# Autodesk Inventor assembly: YIdlePulleyAssembly
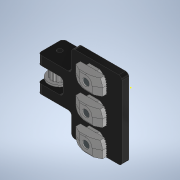
[picture p0: Inventor's stored thumbnail of the model, 180x180]
Saved by Autodesk Inventor 2020.2 (Build 242310000, 310)
## iProperties
Created: 2020-08-24
Part Number: YIdlePulleyAssembly
Document SubType Name: Assembly
Designer: JK
Author: JK
## Documents named in this file (5)
- C:\Users\JK\Documents\Inventor\Anet Upgrade\YIdlePulleyAssembly.iam
- C:\Users\JK\Documents\Inventor\Anet Upgrade\PulleySupport.ipt
- C:\Users\JK\Documents\Inventor\Anet Upgrade\IdlePulley.iam
- C:\Users\JK\Documents\Inventor\Anet Upgrade\T_Slot_Nut_Dropin_3030m5ipt.ipt
- C:\Users\JK\Documents\Inventor\Anet Upgrade\M5x8BoltFlatHead.ipt
## Components (8 placed, 4 different names)
1. PulleySupport:1 — Mate:1, Mate:2, Mate:3, Mate:4, Mate:5, Mate:6, Angle:1, Angle:2, Angle:3, Mate:10, Mate:11, Mate:12
2. IdlePulley:1 [sub-assembly] — Mate:1, Mate:2
3. M5x8BoltFlatHead:1 — Mate:3, Flush:2, Mate:9
4. M5x8BoltFlatHead:2 — Mate:4, Flush:1, Mate:8
5. M5x8BoltFlatHead:3 — Mate:5, Flush:1, Flush:2, Mate:6, Mate:7
6. T_Slot_Nut_Dropin_3030m5ipt:1 — Mate:7, Flush:3, Angle:3
7. T_Slot_Nut_Dropin_3030m5ipt:2 — Mate:8, Flush:3, Flush:4, Angle:1
8. T_Slot_Nut_Dropin_3030m5ipt:3 — Mate:9, Flush:4, Angle:2, Mate:10
## Relationships (19: Mate 12, Flush 4, Angle 3)
- Mate:1: PulleySupport:1 ↔ IdlePulley:1
- Mate:2 (0.2 mm): PulleySupport:1 ↔ IdlePulley:1
- Mate:3: PulleySupport:1 ↔ M5x8BoltFlatHead:1
- Mate:4: PulleySupport:1 ↔ M5x8BoltFlatHead:2
- Mate:5: PulleySupport:1 ↔ M5x8BoltFlatHead:3
- Flush:1: M5x8BoltFlatHead:2 ↔ M5x8BoltFlatHead:3
- Flush:2: M5x8BoltFlatHead:1 ↔ M5x8BoltFlatHead:3
- Mate:6: PulleySupport:1 ↔ M5x8BoltFlatHead:3
- Mate:7: M5x8BoltFlatHead:3 ↔ T_Slot_Nut_Dropin_3030m5ipt:1
- Mate:8: M5x8BoltFlatHead:2 ↔ T_Slot_Nut_Dropin_3030m5ipt:2
- Mate:9: M5x8BoltFlatHead:1 ↔ T_Slot_Nut_Dropin_3030m5ipt:3
- Flush:3: T_Slot_Nut_Dropin_3030m5ipt:1 ↔ T_Slot_Nut_Dropin_3030m5ipt:2
- Flush:4: T_Slot_Nut_Dropin_3030m5ipt:2 ↔ T_Slot_Nut_Dropin_3030m5ipt:3
- Angle:1 (0 deg): PulleySupport:1 ↔ T_Slot_Nut_Dropin_3030m5ipt:2
- Angle:2 (0 deg): PulleySupport:1 ↔ T_Slot_Nut_Dropin_3030m5ipt:3
- Angle:3 (0 deg): PulleySupport:1 ↔ T_Slot_Nut_Dropin_3030m5ipt:1
- Mate:10: PulleySupport:1 ↔ T_Slot_Nut_Dropin_3030m5ipt:3
- Mate:11: PulleySupport:1
- Mate:12 (-10 mm): PulleySupport:1
